# Autodesk Inventor assembly: Motor
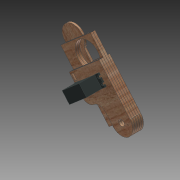
[picture p0: Inventor's stored thumbnail of the model, 180x180]
Saved by Autodesk Inventor 2015 (Build 190159000, 159)
## iProperties
Created: 2015-12-21
Part Number: Motor
Document SubType Name: Assembly
Designer: david
Author: david
## Documents named in this file (9)
- Z:\gip\Inventor\generatie 7\Motor\Motor.iam
- Z:\gip\Inventor\generatie 7\Motor\houder.ipt
- Z:\gip\Inventor\generatie 7\Motor\tanden.ipt
- Z:\gip\Inventor\generatie 7\Motor\servo\block.ipt
- Z:\gip\Inventor\generatie 7\Motor\servo\tang.ipt
- Z:\gip\Inventor\generatie 7\Motor\houder2.ipt
- Z:\gip\Inventor\generatie 7\Motor\houder3.ipt
- Z:\gip\Inventor\generatie 7\Motor\houder4.ipt
- Z:\gip\Inventor\generatie 7\Motor\tandwiel\tandwiel.iam
## Components (10 placed, 8 different names)
1. houder:2 — Mate:19, Flush:3, Flush:4, Flush:26, Mate:25, Flush:27, Flush:31
2. tanden:1 — Mate:32, Angle:1, Mate:45, Mate:46
3. block:1 — Mate:19, Flush:3, Mate:20, Mate:21, Flush:4, Flush:31
4. tang:1 — Mate:20, Mate:21, Mate:42, Mate:44
5. houder2:1 — Flush:26, Mate:25, Flush:27, Mate:26, Flush:28, Mate:27, Mate:43
6. houder3:1 — Mate:26, Flush:28, Mate:27, Flush:30, Mate:30, Mate:31
7. houder3:2 — Flush:30, Mate:30, Mate:31, Mate:32, Angle:1, Mate:37, Flush:32, Mate:38
8. houder4:1 — Mate:37, Flush:32, Mate:38, Flush:33, Mate:39, Mate:40, Mate:45, Mate:46
9. houder:3 — Flush:33, Mate:39, Mate:40
10. tandwiel:1 [sub-assembly] — Mate:42, Mate:43, Mate:44
## Relationships (28: Mate 18, Flush 9, Angle 1)
- Mate:19: houder:2 ↔ block:1
- Flush:3 (-15 mm): houder:2 ↔ block:1
- Mate:20: block:1 ↔ tang:1
- Mate:21: block:1 ↔ tang:1
- Flush:4 (20 mm): houder:2 ↔ block:1
- Flush:26: houder:2 ↔ houder2:1
- Mate:25: houder:2 ↔ houder2:1
- Flush:27: houder:2 ↔ houder2:1
- Mate:26: houder2:1 ↔ houder3:1
- Flush:28: houder2:1 ↔ houder3:1
- Mate:27: houder2:1 ↔ houder3:1
- Flush:30: houder3:1 ↔ houder3:2
- Mate:30: houder3:1 ↔ houder3:2
- Mate:31: houder3:1 ↔ houder3:2
- Mate:32: tanden:1 ↔ houder3:2
- Flush:31 (12.5 mm): houder:2 ↔ block:1
- Angle:1 (0 deg): tanden:1 ↔ houder3:2
- Mate:37: houder3:2 ↔ houder4:1
- Flush:32: houder3:2 ↔ houder4:1
- Mate:38: houder3:2 ↔ houder4:1
- Flush:33: houder4:1 ↔ houder:3
- Mate:39: houder4:1 ↔ houder:3
- Mate:40: houder4:1 ↔ houder:3
- Mate:42: tang:1 ↔ tandwiel:1
- Mate:43: houder2:1 ↔ tandwiel:1
- Mate:44 (0.15 mm): tang:1 ↔ tandwiel:1
- Mate:45: tanden:1 ↔ houder4:1
- Mate:46: tanden:1 ↔ houder4:1
